# Autodesk Inventor assembly: ELEV_000_FULLASMBLY
(part 2 of 2)
- Mate:259: ELEV_013_BAR5(12.000 in):1 ↔ WCP-0897_InlineBearingBlock:6
- Flush:30: ELEV_013_BAR5(12.000 in):1 ↔ WCP-0897_InlineBearingBlock:6
- Mate:260: ELEV_013_BAR5(12.000 in):1 ↔ WCP-0897_InlineBearingBlock:6
- Tangent:3: ELEV_003_BAR3(25.000 in):1 ↔ WCP-0897_InlineBearingBlock:5
- Tangent:4: ELEV_003_BAR3(25.000 in):1 ↔ WCP-0897_InlineBearingBlock:5
- Angle:5 (0 deg): ELEV_003_BAR3(25.000 in):1 ↔ ELEV_013_BAR5(12.000 in):1
- Angle:6 (0 deg): ELEV_003_BAR3(25.000 in):1 ↔ ELEV_013_BAR5(12.000 in):1
- Mate:261: ELEV_013_BAR5(12.000 in):2 ↔ WCP-0897_InlineBearingBlock:7
- Flush:31: ELEV_013_BAR5(12.000 in):2 ↔ WCP-0897_InlineBearingBlock:7
- Mate:262: ELEV_013_BAR5(12.000 in):2 ↔ WCP-0897_InlineBearingBlock:7
- Mate:263: ELEV_013_BAR5(12.000 in):2 ↔ WCP-0897_InlineBearingBlock:8
- Flush:32: ELEV_013_BAR5(12.000 in):2 ↔ WCP-0897_InlineBearingBlock:8
- Mate:264: ELEV_013_BAR5(12.000 in):2 ↔ WCP-0897_InlineBearingBlock:8
- Tangent:5: ELEV_003_BAR3(25.000 in):2 ↔ WCP-0897_InlineBearingBlock:7
- Angle:7 (0 deg): ELEV_004_BAR4(12.000 in):2 ↔ ELEV_013_BAR5(12.000 in):2
- Flush:33: ELEV_003_BAR3(25.000 in):2 ↔ ELEV_013_BAR5(12.000 in):2
- Flush:34: ELEV_013_BAR5(12.000 in):1 ↔ ELEV_013_BAR5(12.000 in):2
- Mate:265: ELEV_003_BAR3(25.000 in):1 ↔ ELEV_011_EXTRUENDCAP:8
- Mate:266: ELEV_003_BAR3(25.000 in):1 ↔ ELEV_011_EXTRUENDCAP:8
- Mate:267: ELEV_003_BAR3(25.000 in):1 ↔ ELEV_011_EXTRUENDCAP:8
- Mate:268: WCP-0897_InlineBearingBlock:8 ↔ COTS_91251A342_Black-Oxide Alloy Steel Socket Head Screw_.5in:9
- Mate:269: WCP-0897_InlineBearingBlock:8 ↔ COTS_91251A342_Black-Oxide Alloy Steel Socket Head Screw_.5in:9
- Mate:270: WCP-0897_InlineBearingBlock:5 ↔ COTS_91251A342_Black-Oxide Alloy Steel Socket Head Screw_.5in:10
- Mate:271: WCP-0897_InlineBearingBlock:5 ↔ COTS_91251A342_Black-Oxide Alloy Steel Socket Head Screw_.5in:10
- Mate:272: WCP-0897_InlineBearingBlock:7 ↔ COTS_91251A342_Black-Oxide Alloy Steel Socket Head Screw_.5in:8
- Mate:273: WCP-0897_InlineBearingBlock:7 ↔ COTS_91251A342_Black-Oxide Alloy Steel Socket Head Screw_.5in:8
- Mate:274: WCP-0897_InlineBearingBlock:6 ↔ COTS_91251A342_Black-Oxide Alloy Steel Socket Head Screw_.5in:7
- Mate:275: WCP-0897_InlineBearingBlock:6 ↔ COTS_91251A342_Black-Oxide Alloy Steel Socket Head Screw_.5in:7
- Mate:276: COTS_91251A342_Black-Oxide Alloy Steel Socket Head Screw_.5in:10 ↔ COTS_90633A411_Low-Strength Steel Thin Nylon-Insert Locknut_10-32:13
- Mate:277: ELEV_013_BAR5(12.000 in):1 ↔ COTS_90633A411_Low-Strength Steel Thin Nylon-Insert Locknut_10-32:13
- Mate:278: COTS_90633A411_Low-Strength Steel Thin Nylon-Insert Locknut_10-32:14 ↔ COTS_91251A342_Black-Oxide Alloy Steel Socket Head Screw_.5in:9
- Mate:279: ELEV_013_BAR5(12.000 in):2 ↔ COTS_90633A411_Low-Strength Steel Thin Nylon-Insert Locknut_10-32:14
- Mate:280: COTS_91251A342_Black-Oxide Alloy Steel Socket Head Screw_.5in:8 ↔ COTS_90633A411_Low-Strength Steel Thin Nylon-Insert Locknut_10-32:15
- Mate:281: ELEV_013_BAR5(12.000 in):2 ↔ COTS_90633A411_Low-Strength Steel Thin Nylon-Insert Locknut_10-32:15
- Mate:282: COTS_90633A411_Low-Strength Steel Thin Nylon-Insert Locknut_10-32:16 ↔ COTS_91251A342_Black-Oxide Alloy Steel Socket Head Screw_.5in:7
- Mate:283: ELEV_013_BAR5(12.000 in):1 ↔ COTS_90633A411_Low-Strength Steel Thin Nylon-Insert Locknut_10-32:16
- Mate:284: ELEV_001_BAR1(27.500 in):1 ↔ ELEV_015_CRSHBLCK1:1
- Mate:285: ELEV_001_BAR1(27.500 in):1 ↔ ELEV_015_CRSHBLCK1:1
- Mate:286: ELEV_001_BAR1(27.500 in):1 ↔ ELEV_015_CRSHBLCK1:1
- Mate:287: ELEV_001_BAR1(27.500 in):2 ↔ ELEV_015_CRSHBLCK1:2
- Mate:288: ELEV_001_BAR1(27.500 in):2 ↔ ELEV_015_CRSHBLCK1:2
- Mate:289: ELEV_001_BAR1(27.500 in):2 ↔ ELEV_015_CRSHBLCK1:2
- Mate:331: COTS_90044A121_Black-Oxide Alloy Steel Socket Head Screw_10-32_2.5in:16 ↔ ELEV_010_BOLTCOVER2:61
- Mate:332: ELEV_012_SUPBRK2_THRD:2 ↔ ELEV_010_BOLTCOVER2:61
- Mate:333: ELEV_013_BAR5(12.000 in):1 ↔ ELEV_011_EXTRUENDCAP:9
- Mate:334: ELEV_013_BAR5(12.000 in):1 ↔ ELEV_011_EXTRUENDCAP:9
- Mate:335: ELEV_013_BAR5(12.000 in):1 ↔ ELEV_011_EXTRUENDCAP:9
- Mate:336: ELEV_013_BAR5(12.000 in):2 ↔ ELEV_011_EXTRUENDCAP:10
- Mate:337: ELEV_013_BAR5(12.000 in):2 ↔ ELEV_011_EXTRUENDCAP:10
- Mate:338: ELEV_013_BAR5(12.000 in):2 ↔ ELEV_011_EXTRUENDCAP:10
- Flush:35: ELEV_001_BAR1(27.500 in):1 ↔ ELEV_019_SUPBAR3:1
- Mate:341: ELEV_001_BAR1(27.500 in):1 ↔ ELEV_019_SUPBAR3:1
- Mate:342: ELEV_019_SUPBAR3:1 ↔ ELEV_019_SUPBAR3:2
- Mate:343: ELEV_019_SUPBAR3:1 ↔ ELEV_019_SUPBAR3:2
- Mate:344: ELEV_019_SUPBAR3:1 ↔ COTS_WCP-0783_1.125ODHexBearing:4
- Mate:345: ELEV_019_SUPBAR3:1 ↔ COTS_WCP-0783_1.125ODHexBearing:2
- Mate:346: ELEV_019_SUPBAR3:2 ↔ COTS_WCP-0783_1.125ODHexBearing:3
- Mate:347: ELEV_019_SUPBAR3:2 ↔ COTS_WCP-0783_1.125ODHexBearing:1
- Mate:348: ELEV_019_SUPBAR3:1 ↔ COTS_WCP-0783_1.125ODHexBearing:4
- Mate:349: ELEV_019_SUPBAR3:1 ↔ COTS_WCP-0783_1.125ODHexBearing:2
- Mate:350: ELEV_019_SUPBAR3:2 ↔ COTS_WCP-0783_1.125ODHexBearing:1
- Mate:351: ELEV_019_SUPBAR3:2 ↔ COTS_WCP-0783_1.125ODHexBearing:3
- Mate:352: COTS_WCP-0783_1.125ODHexBearing:1 ↔ COTS_WCP-0974_#35_15t:1
- Mate:353: COTS_WCP-0783_1.125ODHexBearing:4 ↔ COTS_WCP-0974_#35_15t:2
- Angle:8 (0 deg): COTS_WCP-0783_1.125ODHexBearing:4 ↔ COTS_WCP-0974_#35_15t:2
- Angle:9 (0 deg): COTS_WCP-0783_1.125ODHexBearing:3 ↔ COTS_WCP-0974_#35_15t:2
- Angle:10 (0 deg): COTS_WCP-0783_1.125ODHexBearing:2 ↔ COTS_WCP-0974_#35_15t:1
- Angle:11 (0 deg): COTS_WCP-0783_1.125ODHexBearing:1 ↔ COTS_WCP-0974_#35_15t:1
- Mate:357: ELEV_019_SUPBAR3:1 ↔ ELEV_020_BILLET1(Shit):1
- Mate:358: ELEV_019_SUPBAR3:1 ↔ ELEV_020_BILLET1(Shit):1
- Mate:359: ELEV_001_BAR1(27.500 in):1 ↔ ELEV_020_BILLET1(Shit):1
- Mate:360: ELEV_019_SUPBAR3:2 ↔ ELEV_020_BILLET1(Shit):1
- Mate:361: ELEV_019_SUPBAR3:2 ↔ ELEV_020_BILLET1(Shit):2
- Mate:362: ELEV_019_SUPBAR3:2 ↔ ELEV_020_BILLET1(Shit):2
- Mate:363: ELEV_001_BAR1(27.500 in):2 ↔ ELEV_020_BILLET1(Shit):2
- Mate:364: ELEV_019_SUPBAR3:1 ↔ ELEV_021_SPACER2:5
- Mate:365: ELEV_019_SUPBAR3:1 ↔ ELEV_021_SPACER2:4
- Mate:366: ELEV_019_SUPBAR3:1 ↔ ELEV_021_SPACER2:3
- Mate:367: ELEV_019_SUPBAR3:1 ↔ ELEV_021_SPACER2:2
- Mate:368: ELEV_019_SUPBAR3:1 ↔ ELEV_021_SPACER2:1
- Mate:369: ELEV_019_SUPBAR3:1 ↔ ELEV_021_SPACER2:6
- Mate:370: ELEV_019_SUPBAR3:1 ↔ ELEV_021_SPACER2:6
- Mate:371: ELEV_019_SUPBAR3:1 ↔ ELEV_021_SPACER2:1
- Mate:372: ELEV_019_SUPBAR3:2 ↔ ELEV_021_SPACER2:5
- Mate:373: ELEV_019_SUPBAR3:2 ↔ ELEV_021_SPACER2:4
- Mate:374: ELEV_019_SUPBAR3:1 ↔ ELEV_021_SPACER2:3
- Mate:375: ELEV_019_SUPBAR3:2 ↔ ELEV_021_SPACER2:2
- Mate:376: ELEV_019_SUPBAR3:2 ↔ ELEV_021_SPACER2:3
- Mate:377: COTS_WCP-0974_#35_15t:2 ↔ ELEV_022_WASHER1(3DP):3
- Mate:378: COTS_WCP-0783_1.125ODHexBearing:4 ↔ ELEV_022_WASHER1(3DP):3
- Mate:379: COTS_WCP-0974_#35_15t:2 ↔ ELEV_022_WASHER1(3DP):4
- Mate:380: COTS_WCP-0783_1.125ODHexBearing:2 ↔ ELEV_022_WASHER1(3DP):2
- Mate:381: COTS_WCP-0783_1.125ODHexBearing:2 ↔ ELEV_022_WASHER1(3DP):1
- Mate:382: COTS_WCP-0783_1.125ODHexBearing:2 ↔ ELEV_022_WASHER1(3DP):1
- Mate:383: COTS_WCP-0783_1.125ODHexBearing:1 ↔ ELEV_022_WASHER1(3DP):2
- Mate:384: COTS_WCP-0974_#35_15t:2 ↔ ELEV_022_WASHER1(3DP):4
- Mate:385: COTS_WCP-0974_#35_15t:1 ↔ ELEV_022_WASHER1(3DP):1
- Mate:386: ELEV_019_SUPBAR3:1 ↔ COTS_91251A537_Black-Oxide Alloy Steel Socket Head Screw_.25-20_.5in:1
- Mate:387: ELEV_019_SUPBAR3:1 ↔ COTS_91251A537_Black-Oxide Alloy Steel Socket Head Screw_.25-20_.5in:2
- Mate:388: ELEV_019_SUPBAR3:1 ↔ COTS_91251A537_Black-Oxide Alloy Steel Socket Head Screw_.25-20_.5in:3
- Mate:389: ELEV_019_SUPBAR3:1 ↔ COTS_91251A537_Black-Oxide Alloy Steel Socket Head Screw_.25-20_.5in:4
- Mate:390: ELEV_019_SUPBAR3:1 ↔ COTS_91251A537_Black-Oxide Alloy Steel Socket Head Screw_.25-20_.5in:5
- Mate:391: ELEV_019_SUPBAR3:1 ↔ COTS_91251A537_Black-Oxide Alloy Steel Socket Head Screw_.25-20_.5in:6
- Mate:392: ELEV_019_SUPBAR3:1 ↔ COTS_91251A537_Black-Oxide Alloy Steel Socket Head Screw_.25-20_.5in:5
- Mate:393: ELEV_019_SUPBAR3:1 ↔ COTS_91251A537_Black-Oxide Alloy Steel Socket Head Screw_.25-20_.5in:6
- Mate:394: ELEV_019_SUPBAR3:1 ↔ COTS_91251A537_Black-Oxide Alloy Steel Socket Head Screw_.25-20_.5in:3
- Mate:395: ELEV_019_SUPBAR3:1 ↔ COTS_91251A537_Black-Oxide Alloy Steel Socket Head Screw_.25-20_.5in:4
- Mate:396: ELEV_019_SUPBAR3:1 ↔ COTS_91251A537_Black-Oxide Alloy Steel Socket Head Screw_.25-20_.5in:1
- Mate:397: ELEV_019_SUPBAR3:1 ↔ COTS_91251A537_Black-Oxide Alloy Steel Socket Head Screw_.25-20_.5in:2
- Mate:398: ELEV_019_SUPBAR3:2 ↔ COTS_91251A537_Black-Oxide Alloy Steel Socket Head Screw_.25-20_.5in:11
- Mate:399: ELEV_019_SUPBAR3:2 ↔ COTS_91251A537_Black-Oxide Alloy Steel Socket Head Screw_.25-20_.5in:7
- Mate:400: ELEV_019_SUPBAR3:2 ↔ COTS_91251A537_Black-Oxide Alloy Steel Socket Head Screw_.25-20_.5in:8
- Mate:401: ELEV_019_SUPBAR3:2 ↔ COTS_91251A537_Black-Oxide Alloy Steel Socket Head Screw_.25-20_.5in:9
- Mate:402: ELEV_019_SUPBAR3:2 ↔ COTS_91251A537_Black-Oxide Alloy Steel Socket Head Screw_.25-20_.5in:10
- Mate:403: ELEV_019_SUPBAR3:2 ↔ COTS_91251A537_Black-Oxide Alloy Steel Socket Head Screw_.25-20_.5in:12
- Mate:404: ELEV_019_SUPBAR3:2 ↔ COTS_91251A537_Black-Oxide Alloy Steel Socket Head Screw_.25-20_.5in:11
- Mate:405: ELEV_019_SUPBAR3:2 ↔ COTS_91251A537_Black-Oxide Alloy Steel Socket Head Screw_.25-20_.5in:7
- Mate:406: ELEV_019_SUPBAR3:2 ↔ COTS_91251A537_Black-Oxide Alloy Steel Socket Head Screw_.25-20_.5in:8
- Mate:407: ELEV_019_SUPBAR3:2 ↔ COTS_91251A537_Black-Oxide Alloy Steel Socket Head Screw_.25-20_.5in:9
- Mate:408: ELEV_019_SUPBAR3:2 ↔ COTS_91251A537_Black-Oxide Alloy Steel Socket Head Screw_.25-20_.5in:10
- Mate:409: ELEV_019_SUPBAR3:2 ↔ COTS_91251A537_Black-Oxide Alloy Steel Socket Head Screw_.25-20_.5in:12
- Mate:410: ELEV_019_SUPBAR3:1 ↔ ELEV_023_BILLET2:1
- Mate:411: ELEV_019_SUPBAR3:1 ↔ ELEV_023_BILLET2:1
- Mate:412: ELEV_019_SUPBAR3:1 ↔ ELEV_023_BILLET2:1
- Mate:413: ELEV_019_SUPBAR3:2 ↔ ELEV_023_BILLET2:2
- Mate:414: ELEV_019_SUPBAR3:2 ↔ ELEV_023_BILLET2:2
- Mate:415: ELEV_019_SUPBAR3:1 ↔ ELEV_023_BILLET2:2
- Mate:416: COTS_WCP-0783_1.125ODHexBearing:4 ↔ ELEV_024_SPACER1:1
- Angle:12 (0 deg): COTS_WCP-0783_1.125ODHexBearing:4 ↔ ELEV_024_SPACER1:1
- Flush:36: COTS_WCP-0783_1.125ODHexBearing:4 ↔ ELEV_024_SPACER1:1
- Mate:417: COTS_WCP-0783_1.125ODHexBearing:2 ↔ ELEV_024_SPACER1:2
- Angle:13 (0 deg): COTS_WCP-0783_1.125ODHexBearing:2 ↔ ELEV_024_SPACER1:2
- Flush:37: COTS_WCP-0783_1.125ODHexBearing:2 ↔ ELEV_024_SPACER1:2
## Named parameters: sa_0 = 35585.8
note: some values were not read from the file. Shown as the stored number, unit unknown: "sa_0".
